# Autodesk Inventor assembly: Hanging Rail
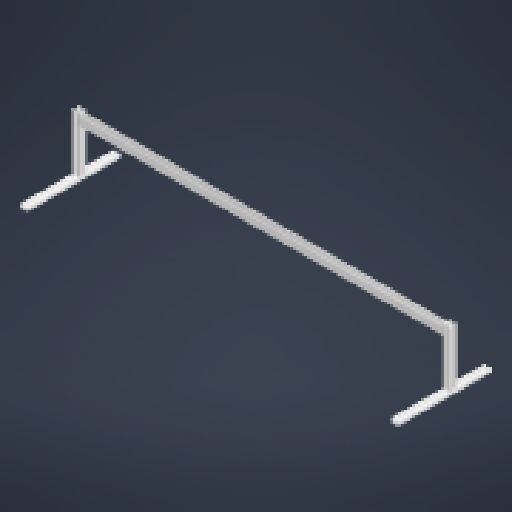
[picture p0: Inventor's stored thumbnail of the model, 512x512]
Saved by Autodesk Inventor 2026.1 (Build 301233020, 233B)
## iProperties
Created: 2025-09-12
Part Number: Hanging Rail
Document SubType Name: Assembly
Designer: atrus
Author: atrus
## Documents named in this file (4)
- C:\Users\atrus\Dropbox\elec\Mechanical\LEDBrick\8020\Hanging Rail.iam
- C:\Users\atrus\Dropbox\elec\Mechanical\LEDBrick\8020\8020-25-2514 X 305.ipt
- C:\Users\atrus\Dropbox\elec\Mechanical\LEDBrick\8020\8020-25-2525 X 180.ipt
- C:\Users\atrus\Dropbox\elec\Mechanical\LEDBrick\8020\8020-25-2503 X 1181_1.ipt
## Components (5 placed, 3 different names)
1. 8020-25-2514 X 305:1 — Mate:1, Flush:1, Flush:5, Flush:6
2. 8020-25-2525 X 180:1 — Mate:1, Flush:1, Flush:2, Mate:2
3. 8020-25-2503 X 1181_1:1 — Flush:2, Mate:2, Flush:4, Mate:4
4. 8020-25-2514 X 305:2 — Mate:3, Flush:3, Flush:5, Flush:6
5. 8020-25-2525 X 180:2 — Mate:3, Flush:3, Flush:4, Mate:4
## Relationships (10: Flush 6, Mate 4)
- Mate:1: 8020-25-2514 X 305:1 ↔ 8020-25-2525 X 180:1
- Flush:1: 8020-25-2514 X 305:1 ↔ 8020-25-2525 X 180:1
- Flush:2: 8020-25-2525 X 180:1 ↔ 8020-25-2503 X 1181_1:1
- Mate:2: 8020-25-2525 X 180:1 ↔ 8020-25-2503 X 1181_1:1
- Mate:3: 8020-25-2514 X 305:2 ↔ 8020-25-2525 X 180:2
- Flush:3: 8020-25-2514 X 305:2 ↔ 8020-25-2525 X 180:2
- Flush:4: 8020-25-2503 X 1181_1:1 ↔ 8020-25-2525 X 180:2
- Mate:4: 8020-25-2503 X 1181_1:1 ↔ 8020-25-2525 X 180:2
- Flush:5: 8020-25-2514 X 305:1 ↔ 8020-25-2514 X 305:2
- Flush:6: 8020-25-2514 X 305:1 ↔ 8020-25-2514 X 305:2
